# Autodesk Inventor assembly: Assieme 2 - Taglio
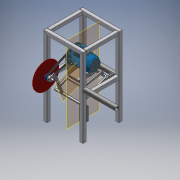
[picture p0: Inventor's stored thumbnail of the model, 180x180]
Saved by Autodesk Inventor 2018 (Build 220112000, 112)
## iProperties
Created: 2020-06-01
Part Number: Assieme 2 - Taglio
Material: Generico
Document SubType Name: Weldment
Designer: Francesco
Weld Material: Welded Aluminum-6061
Author: Francesco
## Documents named in this file (9)
- C:\Users\Francesco\no-brim\Meccanica\Progetto Inventor no-brim\Assiemi\Assieme 2 - Taglio.iam
- C:\Users\Francesco\no-brim\Meccanica\Progetto Inventor no-brim\Assiemi\Telaio - Taglio.iam
- C:\Users\Francesco\no-brim\Meccanica\Progetto Inventor no-brim\Assiemi\Trasmissione cinghie - Taglio.iam
- C:\Users\Francesco\no-brim\Meccanica\Progetto Inventor no-brim\Unificati\it-IT\SKF B - angular contact\SKF B7202 BE.ipt
- C:\Users\Francesco\no-brim\Meccanica\Progetto Inventor no-brim\Parti\Porta cuscinetto perno telaietto.ipt
- C:\Users\Francesco\no-brim\Meccanica\Progetto Inventor no-brim\Parti\Forcella movimento lama.ipt
- C:\Users\Francesco\no-brim\Meccanica\Progetto Inventor no-brim\Parti\Forcella movimento lama 2.ipt
- C:\Users\Francesco\no-brim\Meccanica\Progetto Inventor no-brim\Parti\Perno forcella.ipt
- C:\Users\Francesco\no-brim\Meccanica\Progetto Inventor no-brim\Parti\Pistone salita lama d 40 c 100\AIS2017\536288 ADN-40-100-I-P-A---(0).iam
## Components (10 placed, 7 different names)
1. Telaio - Taglio:1 [sub-assembly] — Coincidente:5, Coincidente:6, Coincidente:7, Coincidente:8, Allineato:1, Allineato:3, Angolo:5, Allineato:12
2. Trasmissione cinghie - Taglio:2 [sub-assembly] — Coincidente:9, Allineato:11, Coincidente:16, Coincidente:17, Angolo:3
3. SKF B- Contatto angolare SKF B7202 BE:1 — Coincidente:1, Coincidente:4, Coincidente:9
4. SKF B- Contatto angolare SKF B7202 BE:2 — Coincidente:2, Coincidente:3
5. Porta cuscinetto perno telaietto:1 — Coincidente:2, Coincidente:3, Coincidente:7, Coincidente:8, Allineato:2
6. Porta cuscinetto perno telaietto:2 — Coincidente:1, Coincidente:4, Coincidente:5, Coincidente:6, Allineato:1, Allineato:2
7. Forcella movimento lama:1 — Coincidente:10, Coincidente:11, Coincidente:18, Coincidente:19, Angolo:4
8. Forcella movimento lama:2 — Coincidente:10, Coincidente:11, Coincidente:14, Coincidente:15, Coincidente:16, Coincidente:17, Angolo:3
9. Perno forcella:1 — Coincidente:14, Coincidente:15
10. 536288 ADN-40-100-I-P-A---(0):1 [sub-assembly] — Coincidente:18, Coincidente:19, Angolo:4, Angolo:5, Allineato:12
## Relationships (25: Mate 17, Flush 5, Angle 3)
- Coincidente:1 [Mate]: SKF B- Contatto angolare SKF B7202 BE:1 ↔ Porta cuscinetto perno telaietto:2
- Coincidente:2 [Mate]: SKF B- Contatto angolare SKF B7202 BE:2 ↔ Porta cuscinetto perno telaietto:1
- Coincidente:3 [Mate]: SKF B- Contatto angolare SKF B7202 BE:2 ↔ Porta cuscinetto perno telaietto:1
- Coincidente:4 [Mate]: SKF B- Contatto angolare SKF B7202 BE:1 ↔ Porta cuscinetto perno telaietto:2
- Coincidente:5 [Mate]: Telaio - Taglio:1 ↔ Porta cuscinetto perno telaietto:2
- Coincidente:6 [Mate] (15 mm): Telaio - Taglio:1 ↔ Porta cuscinetto perno telaietto:2
- Coincidente:7 [Mate]: Telaio - Taglio:1 ↔ Porta cuscinetto perno telaietto:1
- Coincidente:8 [Mate] (15 mm): Telaio - Taglio:1 ↔ Porta cuscinetto perno telaietto:1
- Allineato:1 [Flush] (-2.5 mm): Telaio - Taglio:1 ↔ Porta cuscinetto perno telaietto:2
- Allineato:2 [Flush]: Porta cuscinetto perno telaietto:1 ↔ Porta cuscinetto perno telaietto:2
- Coincidente:9 [Mate]: Trasmissione cinghie - Taglio:2 ↔ SKF B- Contatto angolare SKF B7202 BE:1
- Allineato:3 [Flush] (-225 mm): Telaio - Taglio:1
- Allineato:11 [Flush]: Trasmissione cinghie - Taglio:2
- Coincidente:10 [Mate]: Forcella movimento lama:1 ↔ Forcella movimento lama:2
- Coincidente:11 [Mate]: Forcella movimento lama:1 ↔ Forcella movimento lama:2
- Coincidente:14 [Mate]: Forcella movimento lama:2 ↔ Perno forcella:1
- Coincidente:15 [Mate]: Forcella movimento lama:2 ↔ Perno forcella:1
- Coincidente:16 [Mate]: Trasmissione cinghie - Taglio:2 ↔ Forcella movimento lama:2
- Coincidente:17 [Mate]: Trasmissione cinghie - Taglio:2 ↔ Forcella movimento lama:2
- Angolo:3 [Angle] (0 deg): Trasmissione cinghie - Taglio:2 ↔ Forcella movimento lama:2
- Coincidente:18 [Mate]: Forcella movimento lama:1 ↔ 536288 ADN-40-100-I-P-A---(0):1
- Coincidente:19 [Mate]: Forcella movimento lama:1 ↔ 536288 ADN-40-100-I-P-A---(0):1
- Angolo:4 [Angle] (270 deg): Forcella movimento lama:1 ↔ 536288 ADN-40-100-I-P-A---(0):1
- Angolo:5 [Angle] (0 deg): Telaio - Taglio:1 ↔ 536288 ADN-40-100-I-P-A---(0):1
- Allineato:12 [Flush] (135 mm): Telaio - Taglio:1 ↔ 536288 ADN-40-100-I-P-A---(0):1
